# Autodesk Inventor assembly: 36059
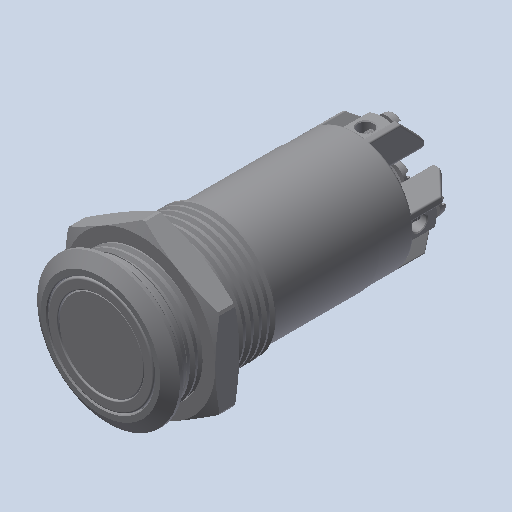
[picture p0: Inventor's stored thumbnail of the model, 512x512]
Saved by Autodesk Inventor 2024.2 (Build 282272000, 272)
## iProperties
Company: TraceParts S.A.
Created: 2020-06-10
Part Number: 36059
Checked By: TraceParts S.A.
Catalog Web Link: www.traceparts.com
Document SubType Name: Assembly
Designer: TraceParts
REFERENCE: 82-4551.1123
SUPPLIER: EAO Switches
RS_STOCK_NUMBER: 8114053
DESIGN: Switch 16mm aluminium 12V blue LED
TIMESTAMP: 20/05/2014 12:05
REVISION: A
TraceParts.PartVersion: 1.0.7
TraceParts.PartStatus: Published
TraceParts.PartLanguage: en
TraceParts.InstanceId: 10-21052014-1176353WPYWGCR5FT74EV57TJFUKWAI
TraceParts.PartTitle: Switch 16mm aluminium 12V blue LED
TRACEPARTS: TRACEPARTS
TraceParts.PartNumber: 10-21052014-117635
TraceParts.ClassPath: RS_COMPONENTS:10-21052014-117635
Author: TraceParts
## Documents named in this file (22)
- C:\Users\lgnds\Documents\GitHub\REACH-Hardware\CAD\InventorProject\Back_Panel\Connectors\82-4551.1123\36059.iam
- C:\Users\lgnds\Documents\GitHub\REACH-Hardware\CAD\InventorProject\Back_Panel\Connectors\82-4551.1123\36059_01.ipt
- C:\Users\lgnds\Documents\GitHub\REACH-Hardware\CAD\InventorProject\Back_Panel\Connectors\82-4551.1123\36059_02.ipt
- C:\Users\lgnds\Documents\GitHub\REACH-Hardware\CAD\InventorProject\Back_Panel\Connectors\82-4551.1123\36059_03.ipt
- C:\Users\lgnds\Documents\GitHub\REACH-Hardware\CAD\InventorProject\Back_Panel\Connectors\82-4551.1123\36059_04.ipt
- C:\Users\lgnds\Documents\GitHub\REACH-Hardware\CAD\InventorProject\Back_Panel\Connectors\82-4551.1123\36059_05.ipt
- C:\Users\lgnds\Documents\GitHub\REACH-Hardware\CAD\InventorProject\Back_Panel\Connectors\82-4551.1123\36059_06.ipt
- C:\Users\lgnds\Documents\GitHub\REACH-Hardware\CAD\InventorProject\Back_Panel\Connectors\82-4551.1123\36059_07.ipt
- C:\Users\lgnds\Documents\GitHub\REACH-Hardware\CAD\InventorProject\Back_Panel\Connectors\82-4551.1123\36059_08.ipt
- C:\Users\lgnds\Documents\GitHub\REACH-Hardware\CAD\InventorProject\Back_Panel\Connectors\82-4551.1123\36059_09.ipt
- C:\Users\lgnds\Documents\GitHub\REACH-Hardware\CAD\InventorProject\Back_Panel\Connectors\82-4551.1123\36059_10.ipt
- C:\Users\lgnds\Documents\GitHub\REACH-Hardware\CAD\InventorProject\Back_Panel\Connectors\82-4551.1123\36059_11.ipt
- C:\Users\lgnds\Documents\GitHub\REACH-Hardware\CAD\InventorProject\Back_Panel\Connectors\82-4551.1123\36059_12.ipt
- C:\Users\lgnds\Documents\GitHub\REACH-Hardware\CAD\InventorProject\Back_Panel\Connectors\82-4551.1123\36059_13.ipt
- C:\Users\lgnds\Documents\GitHub\REACH-Hardware\CAD\InventorProject\Back_Panel\Connectors\82-4551.1123\36059_14.ipt
- C:\Users\lgnds\Documents\GitHub\REACH-Hardware\CAD\InventorProject\Back_Panel\Connectors\82-4551.1123\36059_15.ipt
- C:\Users\lgnds\Documents\GitHub\REACH-Hardware\CAD\InventorProject\Back_Panel\Connectors\82-4551.1123\36059_16.ipt
- C:\Users\lgnds\Documents\GitHub\REACH-Hardware\CAD\InventorProject\Back_Panel\Connectors\82-4551.1123\36059_17.ipt
- C:\Users\lgnds\Documents\GitHub\REACH-Hardware\CAD\InventorProject\Back_Panel\Connectors\82-4551.1123\36059_18.ipt
- C:\Users\lgnds\Documents\GitHub\REACH-Hardware\CAD\InventorProject\Back_Panel\Connectors\82-4551.1123\36059_19.ipt
- C:\Users\lgnds\Documents\GitHub\REACH-Hardware\CAD\InventorProject\Back_Panel\Connectors\82-4551.1123\36059_20.ipt
- C:\Users\lgnds\Documents\GitHub\REACH-Hardware\CAD\InventorProject\Back_Panel\Connectors\82-4551.1123\36059_21.ipt
## Components (21 placed, 21 different names)
1. 36059_01:1
2. 36059_02:1
3. 36059_03:1
4. 36059_04:1
5. 36059_05:1
6. 36059_06:1
7. 36059_07:1
8. 36059_08:1
9. 36059_09:1
10. 36059_10:1
11. 36059_11:1
12. 36059_12:1
13. 36059_13:1
14. 36059_14:1
15. 36059_15:1
16. 36059_16:1
17. 36059_17:1
18. 36059_18:1
19. 36059_19:1 — Rigid:1
20. 36059_20:1 — Rigid:1
21. 36059_21:1
## Relationships (1: WeldJoint 1)
- Rigid:1 [WeldJoint] (3.4 mm): 36059_19:1 ↔ 36059_20:1
